# Autodesk Inventor assembly: Rescuebot 1 en 2
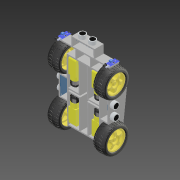
[picture p0: Inventor's stored thumbnail of the model, 180x180]
Saved by Autodesk Inventor 2020.2 (Build 242310000, 310)
## iProperties
Created: 2019-12-09
Part Number: Rescuebot 1 en 2
Document SubType Name: Assembly
Designer: Berkant
Author: Berkant
## Documents named in this file (7)
- C:\Users\berka\Desktop\School\Project 2\Rescuebot ophalen parts\Rescuebot 1 en 2.iam
- C:\Users\berka\Desktop\School\Project 2\Rescuebot ophalen parts\Motorcompartiment.ipt
- C:\Users\berka\Desktop\School\Project 2\Rescuebot ophalen parts\PB en arduino.ipt
- C:\Users\berka\Desktop\School\Project 2\Rescuebot ophalen parts\Arduino Gear Motor.ipt
- C:\Users\berka\Desktop\School\Project 2\Rescuebot ophalen parts\Wiel.ipt
- C:\Users\berka\Desktop\School\Project 2\HC-SR04 Ultrasonic sensor.ipt
- C:\Users\berka\Desktop\ir-sensor.ipt
## Components (15 placed, 6 different names)
1. Motorcompartiment:1 — Rotational:1, Rotational:2, Rotational:3, Rotational:4, Rigid:3, Rigid:4, Rotational:9, Rigid:11, Rigid:12, Rigid:13
2. Arduino Gear Motor:1 — Rotational:4, Rotational:5
3. Arduino Gear Motor:2 — Rotational:2, Rotational:7
4. Arduino Gear Motor:3 — Rotational:3, Rotational:6
5. Arduino Gear Motor:4 — Rotational:1, Rotational:8
6. Wiel:1 — Rotational:8
7. Wiel:2 — Rotational:7
8. Wiel:3 — Rotational:6
9. Wiel:4 — Rotational:5
10. HC-SR04 Ultrasonic sensor:3 — Rigid:3
11. PB en arduino:1 — Rigid:4
12. HC-SR04 Ultrasonic sensor:4 — Rigid:11
13. HC-SR04 Ultrasonic sensor:6 — Rotational:9
14. ir-sensor:1 — Rigid:12
15. ir-sensor:2 — Rigid:13
## Relationships (14: RevoluteJoint 9, WeldJoint 5)
- Rotational:1 [RevoluteJoint]: Motorcompartiment:1 ↔ Arduino Gear Motor:4
- Rotational:2 [RevoluteJoint]: Motorcompartiment:1 ↔ Arduino Gear Motor:2
- Rotational:3 [RevoluteJoint]: Motorcompartiment:1 ↔ Arduino Gear Motor:3
- Rotational:4 [RevoluteJoint]: Motorcompartiment:1 ↔ Arduino Gear Motor:1
- Rotational:5 [RevoluteJoint] (3 mm): Arduino Gear Motor:1 ↔ Wiel:4
- Rotational:6 [RevoluteJoint] (3 mm): Arduino Gear Motor:3 ↔ Wiel:3
- Rotational:7 [RevoluteJoint] (3 mm): Arduino Gear Motor:2 ↔ Wiel:2
- Rotational:8 [RevoluteJoint] (3 mm): Arduino Gear Motor:4 ↔ Wiel:1
- Rigid:3 [WeldJoint]: Motorcompartiment:1 ↔ HC-SR04 Ultrasonic sensor:3
- Rigid:4 [WeldJoint]: Motorcompartiment:1 ↔ PB en arduino:1
- Rotational:9 [RevoluteJoint]: Motorcompartiment:1 ↔ HC-SR04 Ultrasonic sensor:6
- Rigid:11 [WeldJoint]: Motorcompartiment:1 ↔ HC-SR04 Ultrasonic sensor:4
- Rigid:12 [WeldJoint] (1 mm): Motorcompartiment:1 ↔ ir-sensor:1
- Rigid:13 [WeldJoint] (1 mm): Motorcompartiment:1 ↔ ir-sensor:2
